# Autodesk Inventor assembly: 下半身_6
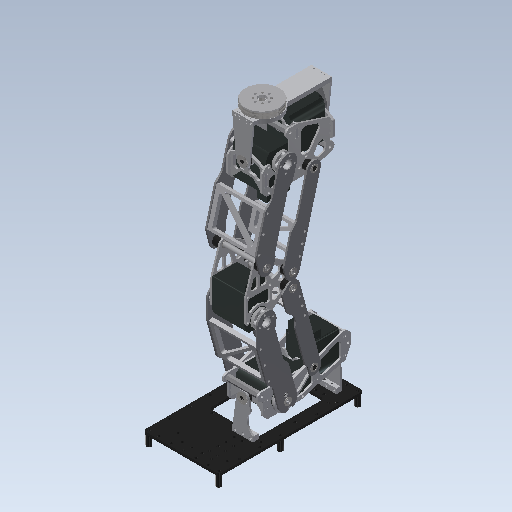
[picture p0: Inventor's stored thumbnail of the model, 512x512]
Saved by Autodesk Inventor 2020.3 (Build 243373000, 373)
## iProperties
Created: 2016-08-23
Part Number: 下半身_6
Material: 一般
Document SubType Name: Assembly
Designer: hiro
Mass: 967.04 g
Surface Area: 2501.85 cm^2
Volume: 430.712 cm^3
Density: 2.24521 g/cm^3
Author: hiro
## Documents named in this file (14)
- C:\Users\masato\Documents\Inventor\CITBrains\スペーサー\OpenPlatform_ver3_0\下半身_6_MIR.iam
- C:\Users\masato\Documents\Inventor\CITBrains\スペーサー\OpenPlatform_ver3_0\下半身\足首\足首_独立ピッチ_1.iam
- C:\Users\masato\Documents\Inventor\CITBrains\スペーサー\OpenPlatform_ver3_0\下半身_160823\リンク\リンク_6_2.iam
- C:\Users\masato\Documents\Inventor\CITBrains\スペーサー\OpenPlatform_ver3_0\下半身_160823\リンク\リンク_6_3.iam
- C:\Users\masato\Documents\Inventor\CITBrains\スペーサー\OpenPlatform_ver3_0\下半身_160823\リンク\リンク_6_4.iam
- C:\Users\masato\Documents\Inventor\CITBrains\スペーサー\OpenPlatform_ver3_0\下半身_160823\付け根ロール\付け根ロール_1.iam
- C:\Users\masato\Documents\Inventor\CITBrains\スペーサー\OpenPlatform_ver3_0\下半身_160823\付け根ロール\長穴減速_ホーン_2.iam
- C:\Users\masato\Documents\Inventor\CITBrains\スペーサー\OpenPlatform_ver3_0\下半身_160823\リンク\長穴減速_ホーン_2.iam
- C:\Users\masato\Documents\Inventor\CITBrains\スペーサー\OpenPlatform_ver3_0\下半身\足裏\足裏_1_1_MIR.iam
- C:\Users\masato\Documents\Inventor\CITBrains\スペーサー\OpenPlatform_ver3_0\下半身_160823\膝\膝_6_1_MIR.iam
- C:\Users\masato\Documents\Inventor\CITBrains\スペーサー\OpenPlatform_ver3_0\下半身_160823\付け根\付け根_1_MIR.iam
- C:\Users\masato\Documents\Inventor\CITBrains\スペーサー\OpenPlatform_ver3_0\下半身_160823\リンク\リンク_ふくらはぎ_サブフレーム_1_4.ipt
- C:\Users\masato\Documents\Inventor\CITBrains\スペーサー\OpenPlatform_ver3_0\下半身\足首\足首_1_MIR.iam
- C:\Users\masato\Documents\Inventor\CITBrains\スペーサー\OpenPlatform_ver3_0\下半身_160823\リンク\リンク_6_1.iam
## Components (16 placed, 12 different names)
1. 付け根ロール_1:1 [sub-assembly] — メイト:23, フラッシュ:25, フラッシュ:26, 角度:23, 角度:24, 円柱状:1, 角度:33, 挿入:103
2. 足首_独立ピッチ_1:1 [sub-assembly] — 挿入:87, 挿入:100, 挿入:102
3. 長穴減速_ホーン_2:1 [sub-assembly] — 挿入:46, 挿入:104
4. リンク_6_4:1 [sub-assembly] — 角度:18, 角度:19, 角度:20, 角度:21, 挿入:82, 挿入:105
5. リンク_6_2:1 [sub-assembly] — 角度:14, 角度:15, 角度:17, 挿入:86, 挿入:87, 角度:32
6. 長穴減速_ホーン_2:2 [sub-assembly] — 挿入:46, 円柱状:1
7. 足裏_1_1_MIR:1 [sub-assembly] — 角度:33, 挿入:101
8. 膝_6_1_MIR:1 [sub-assembly] — 角度:20, 角度:18, 角度:14, 角度:15, 角度:19, 角度:17, 角度:21, 挿入:76, 挿入:77, 挿入:78, 挿入:79, 挿入:82, 挿入:84, 角度:30, 角度:32, 挿入:99
9. 付け根_1_MIR:1 [sub-assembly] — 角度:23, 角度:24, 挿入:103, 挿入:104, 挿入:106, 挿入:107, 挿入:108, 挿入:109, 挿入:110
10. リンク_ふくらはぎ_サブフレーム_1_4:1 — 挿入:108, 挿入:109
11. リンク_ふくらはぎ_サブフレーム_1_4:2 — 挿入:105, 挿入:106, 挿入:107
12. リンク_ふくらはぎ_サブフレーム_1_4:3 — 挿入:78, 挿入:79, 挿入:86
13. リンク_ふくらはぎ_サブフレーム_1_4:4 — 挿入:76, 挿入:77
14. リンク_6_3:2 [sub-assembly] — 挿入:84, 挿入:110
15. 足首_1_MIR:1 [sub-assembly] — 角度:30, 挿入:101, 挿入:102
16. リンク_6_1:1 [sub-assembly] — 挿入:99, 挿入:100
## Relationships (37: Insert 21, Angle 12, Flush 2, Mate 1, CylindricalJoint 1)
- 角度:14 [Angle] (0 deg): リンク_6_2:1 ↔ 膝_6_1_MIR:1
- 角度:15 [Angle] (-30 deg): リンク_6_2:1 ↔ 膝_6_1_MIR:1
- 角度:17 [Angle] (90 deg): リンク_6_2:1 ↔ 膝_6_1_MIR:1
- 角度:18 [Angle] (0 deg): リンク_6_4:1 ↔ 膝_6_1_MIR:1
- 角度:19 [Angle] (30 deg): リンク_6_4:1 ↔ 膝_6_1_MIR:1
- 角度:20 [Angle] (15 deg): リンク_6_4:1 ↔ 膝_6_1_MIR:1
- 角度:21 [Angle] (90 deg): リンク_6_4:1 ↔ 膝_6_1_MIR:1
- メイト:23 [Mate]: 付け根ロール_1:1
- フラッシュ:25 [Flush]: 付け根ロール_1:1
- フラッシュ:26 [Flush]: 付け根ロール_1:1
- 挿入:46 [Insert]: 長穴減速_ホーン_2:1 ↔ 長穴減速_ホーン_2:2
- 角度:23 [Angle] (45 deg): 付け根ロール_1:1 ↔ 付け根_1_MIR:1
- 角度:24 [Angle] (20 deg): 付け根ロール_1:1 ↔ 付け根_1_MIR:1
- 挿入:76 [Insert]: 膝_6_1_MIR:1 ↔ リンク_ふくらはぎ_サブフレーム_1_4:4
- 挿入:77 [Insert]: 膝_6_1_MIR:1 ↔ リンク_ふくらはぎ_サブフレーム_1_4:4
- 挿入:78 [Insert]: 膝_6_1_MIR:1 ↔ リンク_ふくらはぎ_サブフレーム_1_4:3
- 挿入:79 [Insert]: 膝_6_1_MIR:1 ↔ リンク_ふくらはぎ_サブフレーム_1_4:3
- 挿入:82 [Insert]: リンク_6_4:1 ↔ 膝_6_1_MIR:1
- 挿入:84 [Insert]: 膝_6_1_MIR:1 ↔ リンク_6_3:2
- 挿入:86 [Insert]: リンク_6_2:1 ↔ リンク_ふくらはぎ_サブフレーム_1_4:3
- 挿入:87 [Insert]: 足首_独立ピッチ_1:1 ↔ リンク_6_2:1
- 円柱状:1 [CylindricalJoint]: 付け根ロール_1:1 ↔ 長穴減速_ホーン_2:2
- 角度:30 [Angle] (0 deg): 膝_6_1_MIR:1 ↔ 足首_1_MIR:1
- 角度:32 [Angle] (-15 deg): リンク_6_2:1 ↔ 膝_6_1_MIR:1
- 挿入:99 [Insert]: 膝_6_1_MIR:1 ↔ リンク_6_1:1
- 挿入:100 [Insert]: 足首_独立ピッチ_1:1 ↔ リンク_6_1:1
- 角度:33 [Angle] (180 deg): 付け根ロール_1:1 ↔ 足裏_1_1_MIR:1
- 挿入:101 [Insert]: 足裏_1_1_MIR:1 ↔ 足首_1_MIR:1
- 挿入:102 [Insert]: 足首_独立ピッチ_1:1 ↔ 足首_1_MIR:1
- 挿入:103 [Insert]: 付け根ロール_1:1 ↔ 付け根_1_MIR:1
- 挿入:104 [Insert]: 長穴減速_ホーン_2:1 ↔ 付け根_1_MIR:1
- 挿入:105 [Insert]: リンク_6_4:1 ↔ リンク_ふくらはぎ_サブフレーム_1_4:2
- 挿入:106 [Insert]: 付け根_1_MIR:1 ↔ リンク_ふくらはぎ_サブフレーム_1_4:2
- 挿入:107 [Insert]: 付け根_1_MIR:1 ↔ リンク_ふくらはぎ_サブフレーム_1_4:2
- 挿入:108 [Insert]: 付け根_1_MIR:1 ↔ リンク_ふくらはぎ_サブフレーム_1_4:1
- 挿入:109 [Insert]: 付け根_1_MIR:1 ↔ リンク_ふくらはぎ_サブフレーム_1_4:1
- 挿入:110 [Insert]: 付け根_1_MIR:1 ↔ リンク_6_3:2
## Named parameters: sa_0 = 80000, sa_1 = -5.398e-10, sa_2 = 3.965e-10
note: some values were not read from the file. Shown as the stored number, unit unknown: "sa_0", "sa_1", "sa_2".
